# Autodesk Inventor assembly: ResistojetPrototype
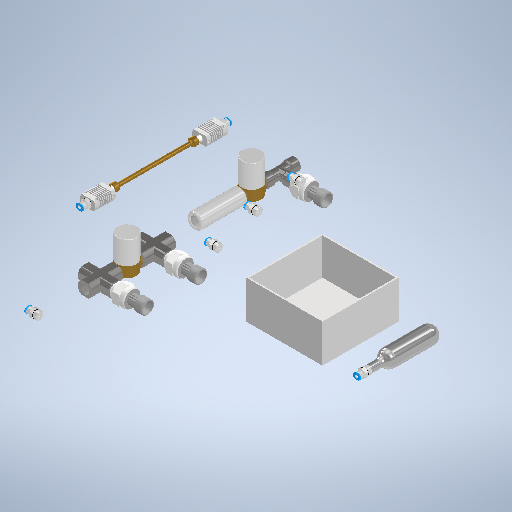
[picture p0: Inventor's stored thumbnail of the model, 512x512]
Saved by Autodesk Inventor 2025.2 (Build 292293000, 293)
## iProperties
Created: 2026-06-11
Part Number: ResistojetPrototype
Document SubType Name: Assembly
Designer: Simon
Author: Simon
## Documents named in this file (12)
- C:\Users\Simon\Projects\MEng Electronics\Development of a Resistojet Thruster\3) Hardware\Resistojet Design\Prototype Design\ResistojetPrototype.iam
- C:\Users\Simon\Projects\MEng Electronics\Development of a Resistojet Thruster\3) Hardware\Resistojet Design\Prototype Design\Heater.ipt
- C:\Users\Simon\Projects\MEng Electronics\Development of a Resistojet Thruster\3) Hardware\Resistojet Design\Prototype Design\PressureSensor.ipt
- C:\Users\Simon\Projects\MEng Electronics\Development of a Resistojet Thruster\3) Hardware\Resistojet Design\Prototype Design\SolenoidValve.ipt
- C:\Users\Simon\Projects\MEng Electronics\Development of a Resistojet Thruster\3) Hardware\Resistojet Design\Prototype Design\Plenum.ipt
- C:\Users\Simon\Projects\MEng Electronics\Development of a Resistojet Thruster\3) Hardware\Resistojet Design\Prototype Design\0,250' NPT TEE.ipt
- C:\Users\Simon\Projects\MEng Electronics\Development of a Resistojet Thruster\3) Hardware\Resistojet Design\Prototype Design\1-4 NPT 4 Way Cross Pneumatic Fitting.ipt
- C:\Users\Simon\Projects\MEng Electronics\Development of a Resistojet Thruster\3) Hardware\Resistojet Design\Prototype Design\BicycleTank.ipt
- C:\Users\Simon\Projects\MEng Electronics\Development of a Resistojet Thruster\3) Hardware\Resistojet Design\Prototype Design\Festo_Pneumatic_Coupling_PC4-M10.ipt
- C:\Users\Simon\Projects\MEng Electronics\Development of a Resistojet Thruster\3) Hardware\Resistojet Design\Prototype Design\Box.ipt
- C:\Users\Simon\Projects\MEng Electronics\Development of a Resistojet Thruster\3) Hardware\Resistojet Design\Prototype Design\Creality Heatsink v1.2.ipt
- C:\Users\Simon\Projects\MEng Electronics\Development of a Resistojet Thruster\3) Hardware\Resistojet Design\Prototype Design\Heatbreak CR30.ipt
## Components (23 placed, 11 different names)
1. Heater:1 — Mate:35, Mate:36, Mate:43, Mate:44
2. PressureSensor:1 — Mate:16, Mate:25
3. PressureSensor:2 — Mate:6, Mate:8
4. PressureSensor:3 — Mate:19, Mate:26
5. SolenoidValve:1 — Mate:5, Flush:1, Mate:7, Mate:9, Mate:10
6. SolenoidValve:2 — Flush:1, Mate:15, Mate:18, Mate:23, Mate:24
7. Plenum:1 — Mate:9, Mate:10
8. 0,250' NPT TEE:1 — Mate:5, Mate:6, Mate:7, Mate:8
9. 1-4 NPT 4 Way Cross Pneumatic Fitting:1 — Mate:15, Mate:16, Mate:24, Mate:25
10. 1-4 NPT 4 Way Cross Pneumatic Fitting:2 — Mate:18, Mate:19, Mate:23, Mate:26
11. BicycleTank:1
12. Festo_Pneumatic_Coupling_PC4-M10:1
13. Festo_Pneumatic_Coupling_PC4-M10:2
14. Festo_Pneumatic_Coupling_PC4-M10:3
15. Festo_Pneumatic_Coupling_PC4-M10:4 — Mate:37, Mate:38
16. Festo_Pneumatic_Coupling_PC4-M10:5
17. Festo_Pneumatic_Coupling_PC4-M10:6
18. Box:1
19. Creality Heatsink v1.2:1 — Mate:33, Mate:34, Mate:37, Mate:38
20. Heatbreak CR30:1 — Mate:33, Mate:34, Mate:35, Mate:36
21. Festo_Pneumatic_Coupling_PC4-M10:7
22. Creality Heatsink v1.2:2
23. Heatbreak CR30:2 — Mate:43, Mate:44
## Relationships (27: Mate 26, Flush 1)
- Mate:5: SolenoidValve:1 ↔ 0,250' NPT TEE:1
- Mate:6: PressureSensor:2 ↔ 0,250' NPT TEE:1
- Flush:1: SolenoidValve:1 ↔ SolenoidValve:2
- Mate:7 (-10 mm): SolenoidValve:1 ↔ 0,250' NPT TEE:1
- Mate:8 (-7 mm): PressureSensor:2 ↔ 0,250' NPT TEE:1
- Mate:9: SolenoidValve:1 ↔ Plenum:1
- Mate:10 (-10 mm): SolenoidValve:1 ↔ Plenum:1
- Mate:15: SolenoidValve:2 ↔ 1-4 NPT 4 Way Cross Pneumatic Fitting:1
- Mate:16: PressureSensor:1 ↔ 1-4 NPT 4 Way Cross Pneumatic Fitting:1
- Mate:18: SolenoidValve:2 ↔ 1-4 NPT 4 Way Cross Pneumatic Fitting:2
- Mate:19: PressureSensor:3 ↔ 1-4 NPT 4 Way Cross Pneumatic Fitting:2
- Mate:23 (-10 mm): SolenoidValve:2 ↔ 1-4 NPT 4 Way Cross Pneumatic Fitting:2
- Mate:24 (-10 mm): SolenoidValve:2 ↔ 1-4 NPT 4 Way Cross Pneumatic Fitting:1
- Mate:25 (-7 mm): PressureSensor:1 ↔ 1-4 NPT 4 Way Cross Pneumatic Fitting:1
- Mate:26 (-7 mm): PressureSensor:3 ↔ 1-4 NPT 4 Way Cross Pneumatic Fitting:2
- Mate:33: Creality Heatsink v1.2:1 ↔ Heatbreak CR30:1
- Mate:34: Creality Heatsink v1.2:1 ↔ Heatbreak CR30:1
- Mate:35: Heater:1 ↔ Heatbreak CR30:1
- Mate:36: Heater:1 ↔ Heatbreak CR30:1
- Mate:37: Festo_Pneumatic_Coupling_PC4-M10:4 ↔ Creality Heatsink v1.2:1
- Mate:38: Festo_Pneumatic_Coupling_PC4-M10:4 ↔ Creality Heatsink v1.2:1
- [Mate]: Creality Heatsink v1.2:2 ↔ Heatbreak CR30:2
- [Mate]: Creality Heatsink v1.2:2 ↔ Heatbreak CR30:2
- [Mate]: Festo_Pneumatic_Coupling_PC4-M10:7 ↔ Creality Heatsink v1.2:2
- [Mate]: Festo_Pneumatic_Coupling_PC4-M10:7 ↔ Creality Heatsink v1.2:2
- Mate:43: Heater:1 ↔ Heatbreak CR30:2
- Mate:44: Heater:1 ↔ Heatbreak CR30:2
## Named parameters: d43_d37 = 0 mm, d44_d38 = 0 mm, d45_d41 = 0 mm, d46_d42 = 0 mm
